# Autodesk Inventor assembly: PCB_hub_rev_0
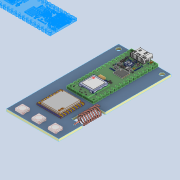
[picture p0: Inventor's stored thumbnail of the model, 180x180]
Saved by Autodesk Inventor 2022 (Build 260153000, 153)
## iProperties
Company: Open CASCADE
Created: 2025-09-22
Part Number: PCB_hub_rev_0
Description: Designed by EasyEDA Pro
Document SubType Name: Assembly
Designer: 1234
Authority: Unknown
Sending System: Open CASCADE 7.8
Preprocessor: Open CASCADE STEP processor 7.8
Title: Open CASCADE Shape Model
Author: Author
## Documents named in this file (9)
- C:\Users\1234\Dropbox\Giorgio_Mac\PPS (pascon piccone sacchiero)\PCB\PCB_hub_rev_0\PCB_hub_rev_0.iam
- C:\Users\1234\Dropbox\Giorgio_Mac\PPS (pascon piccone sacchiero)\PCB\PCB_hub_rev_0\Board~ZvB2.ipt
- C:\Users\1234\Dropbox\Giorgio_Mac\PPS (pascon piccone sacchiero)\PCB\PCB_hub_rev_0\U2~Arduino_NANO_ESP32~libraries_Arduino_NANO_ESP32.step~ZvB2.iam
- C:\Users\1234\Dropbox\Giorgio_Mac\PPS (pascon piccone sacchiero)\PCB\PCB_hub_rev_0\C6~C1206~C1206_L3.2-W1.6-H1.3~ZvB2.iam
- C:\Users\1234\Dropbox\Giorgio_Mac\PPS (pascon piccone sacchiero)\PCB\PCB_hub_rev_0\C4~C0603~C0603_L1.6-W0.8-H0.8~ZvB2.iam
- C:\Users\1234\Dropbox\Giorgio_Mac\PPS (pascon piccone sacchiero)\PCB\PCB_hub_rev_0\LD1~LED-SMD_4P-L5.0-W5.0-BL_XL-5050RGBC~LED-SMD_4P-L5.0-W5.0-BL_XL-5050RGBC~ZvB2.iam
- C:\Users\1234\Dropbox\Giorgio_Mac\PPS (pascon piccone sacchiero)\PCB\PCB_hub_rev_0\U1~SOT-223-3_L6.5-W3.4-P2.30-LS7.0-BR-1~SOT-223-3_L6.5-W3.4-P2.30-LS7.0-BR-1~ZvB2.iam
- C:\Users\1234\Dropbox\Giorgio_Mac\PPS (pascon piccone sacchiero)\PCB\PCB_hub_rev_0\U3~COMM-SMD_LORA1276-C1-915MHZ~COMM-SMD_LORA1276-C1-915MHZ~ZvB2.iam
- C:\Users\1234\Dropbox\Giorgio_Mac\PPS (pascon piccone sacchiero)\PCB\PCB_hub_rev_0\ANT1~ANT-TH_VG868SNX18-5W2~ANT-TH_VG868SNX18-5W2~ZvB2.iam
## Components (14 placed, 14 different names)
1. Board~ZvB2_1 — Mate:1, Flush:1
2. U2~Arduino_NANO_ESP32~libraries\Arduino_NANO_ESP32.step~ZvB2_190 [sub-assembly] — Mate:1, Flush:1
3. C6~C1206~C1206_L3.2-W1.6-H1.3~ZvB2_192 [sub-assembly]
4. C6~C1206~C1206_L3.2-W1.6-H1.3~ZvB2_193 [sub-assembly]
5. C6~C1206~C1206_L3.2-W1.6-H1.3~ZvB2_194 [sub-assembly]
6. C4~C0603~C0603_L1.6-W0.8-H0.8~ZvB2_196 [sub-assembly]
7. C4~C0603~C0603_L1.6-W0.8-H0.8~ZvB2_197 [sub-assembly]
8. C4~C0603~C0603_L1.6-W0.8-H0.8~ZvB2_198 [sub-assembly]
9. LD1~LED-SMD_4P-L5.0-W5.0-BL_XL-5050RGBC~LED-SMD_4P-L5.0-W5.0-BL_XL-5050RGBC~ZvB2_200 [sub-assembly]
10. LD1~LED-SMD_4P-L5.0-W5.0-BL_XL-5050RGBC~LED-SMD_4P-L5.0-W5.0-BL_XL-5050RGBC~ZvB2_201 [sub-assembly]
11. LD1~LED-SMD_4P-L5.0-W5.0-BL_XL-5050RGBC~LED-SMD_4P-L5.0-W5.0-BL_XL-5050RGBC~ZvB2_202 [sub-assembly]
12. U1~SOT-223-3_L6.5-W3.4-P2.30-LS7.0-BR-1~SOT-223-3_L6.5-W3.4-P2.30-LS7.0-BR-1~ZvB2_204 [sub-assembly]
13. U3~COMM-SMD_LORA1276-C1-915MHZ~COMM-SMD_LORA1276-C1-915MHZ~ZvB2_206 [sub-assembly]
14. ANT1~ANT-TH_VG868SNX18-5W2~ANT-TH_VG868SNX18-5W2~ZvB2_208 [sub-assembly]
## Relationships (2: Mate 1, Flush 1)
- Mate:1: Board~ZvB2_1 ↔ U2~Arduino_NANO_ESP32~libraries\Arduino_NANO_ESP32.step~ZvB2_190
- Flush:1: Board~ZvB2_1 ↔ U2~Arduino_NANO_ESP32~libraries\Arduino_NANO_ESP32.step~ZvB2_190
